# Autodesk Inventor assembly: LEG_MIR_MIR1
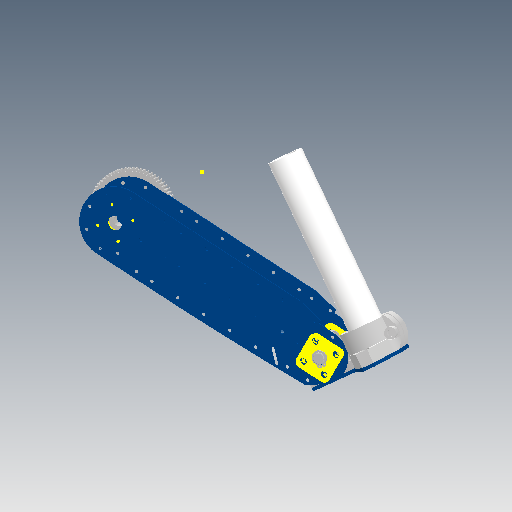
[picture p0: Inventor's stored thumbnail of the model, 512x512]
Saved by Autodesk Inventor 2020.5 (Build 245400000, 400)
## iProperties
Created: 2022-10-31
Part Number: LEG_MIR_MIR1
Document SubType Name: Assembly
Designer: kanazawakotaro
Author: Administrator
## Documents named in this file (12)
- C:\Users\Administrator\Documents\kamuy2\kamuy2\LEG_MIR_MIR1.iam
- C:\Users\Administrator\Documents\kamuy2\kamuy2\Parts\Part2_MIR_MIR_MIR1.ipt
- C:\Users\Administrator\Documents\kamuy2\kamuy2\Parts\GEABP1.0-70-10-A-19-KFC30-K3_Autodesk_Inventor_2020_20221114\AIS2020\GEABP1_0-70-10-A-19-KFC30-K3_MIR_MIR_MIR1.iam
- C:\Users\Administrator\Documents\kamuy2\kamuy2\Parts\PIJX30-20-150_Autodesk_Inventor_2020_20221115\PIJX30-20-150_MIR_MIR_MIR1.ipt
- C:\Users\Administrator\Documents\kamuy2\kamuy2\Parts\C-SHA10_Autodesk_Inventor_2020_20221104\AIS2020\C-SHA10_MIR_MIR_MIR1.iam
- C:\Users\Administrator\Documents\kamuy2\kamuy2\Part16_MIR_MIR_MIR1.ipt
- C:\Users\Administrator\Documents\kamuy2\kamuy2\Parts\HTPA30S3M060-A-N10_Autodesk_Inventor_2020_20221115\AIS2020\HTPA30S3M060-A-N10_MIR_MIR_MIR1.iam
- C:\Users\Administrator\Documents\kamuy2\kamuy2\Part20_MIR_MIR_MIR1.ipt
- C:\Users\Administrator\Documents\kamuy2\kamuy2\Parts\SMYHF30_STEP_AP203AP214\SMYHF30_203_MIR_MIR_MIR1.ipt
- C:\Users\Administrator\Documents\kamuy2\kamuy2\Part22_MIR_MIR_MIR1.ipt
- C:\Users\Administrator\Documents\kamuy2\kamuy2\Parts\RORPOS20-L30_Autodesk_Inventor_2020_20221117\AIS2020\RORPOS20-L30_MIR_MIR_MIR1.iam
- C:\Users\Administrator\Documents\kamuy2\kamuy2\Parts\NSFMRRA10-74-B3-S3-KC31.5-A11_Autodesk_Inventor_2020_20221116\AIS2020\NSFMRRA10-74-B3-S3-KC31_5-A11(000_000)_MIR_MIR_MIR1.iam
## Components (16 placed, 11 different names)
1. Part2_MIR_MIR_MIR1:1
2. GEABP1_0-70-10-A-19-KFC30-K3_MIR_MIR_MIR1:1 [sub-assembly] — フラッシュ:123
3. PIJX30-20-150_MIR_MIR_MIR1:1 — メイト:244, メイト:245
4. C-SHA10_MIR_MIR_MIR1:1 [sub-assembly] — フラッシュ:131, フラッシュ:89, メイト:235, メイト:249, フラッシュ:133, メイト:264
5. C-SHA10_MIR_MIR_MIR1:2 [sub-assembly] — フラッシュ:131, フラッシュ:89, メイト:237, メイト:250
6. Part16_MIR_MIR_MIR1:1 — フラッシュ:96, フラッシュ:122, メイト:236
7. Part16_MIR_MIR_MIR1:2 — フラッシュ:96, メイト:219, メイト:164, メイト:230
8. Part16_MIR_MIR_MIR1:3 — フラッシュ:122, メイト:219, メイト:234, フラッシュ:139, メイト:252
9. HTPA30S3M060-A-N10_MIR_MIR_MIR1:1 [sub-assembly] — フラッシュ:138, メイト:263
10. HTPA30S3M060-A-N10_MIR_MIR_MIR1:2 [sub-assembly] — フラッシュ:138, メイト:164
11. Part20_MIR_MIR_MIR1:1 — メイト:237, メイト:236, フラッシュ:123, メイト:265, メイト:66, メイト:68
12. Part20_MIR_MIR_MIR1:2 — メイト:265, メイト:235, メイト:234, メイト:230, メイト:251, メイト:247, メイト:253, メイト:69
13. SMYHF30_203_MIR_MIR_MIR1:1 — メイト:244, メイト:246, フラッシュ:135, メイト:242
14. Part22_MIR_MIR_MIR1:1 — メイト:250, メイト:249, メイト:246, フラッシュ:135, メイト:245, メイト:242, フラッシュ:133
15. RORPOS20-L30_MIR_MIR_MIR1:1 [sub-assembly] — メイト:251, メイト:247
16. NSFMRRA10-74-B3-S3-KC31_5-A11(000_000)_MIR_MIR_MIR1:1 [sub-assembly] — メイト:264, メイト:263, メイト:253, フラッシュ:139, メイト:252, メイト:66, メイト:68, メイト:69
## Relationships (32: Mate 25, Flush 7)
- フラッシュ:131 [Flush]: C-SHA10_MIR_MIR_MIR1:1 ↔ C-SHA10_MIR_MIR_MIR1:2
- フラッシュ:89 [Flush]: C-SHA10_MIR_MIR_MIR1:1 ↔ C-SHA10_MIR_MIR_MIR1:2
- フラッシュ:96 [Flush]: Part16_MIR_MIR_MIR1:1 ↔ Part16_MIR_MIR_MIR1:2
- フラッシュ:122 [Flush]: Part16_MIR_MIR_MIR1:1 ↔ Part16_MIR_MIR_MIR1:3
- メイト:219 [Mate] (168 mm): Part16_MIR_MIR_MIR1:2 ↔ Part16_MIR_MIR_MIR1:3
- フラッシュ:138 [Flush]: HTPA30S3M060-A-N10_MIR_MIR_MIR1:1 ↔ HTPA30S3M060-A-N10_MIR_MIR_MIR1:2
- メイト:164 [Mate] (7 mm): Part16_MIR_MIR_MIR1:2 ↔ HTPA30S3M060-A-N10_MIR_MIR_MIR1:2
- メイト:237 [Mate] (6 mm): C-SHA10_MIR_MIR_MIR1:2 ↔ Part20_MIR_MIR_MIR1:1
- メイト:236 [Mate]: Part16_MIR_MIR_MIR1:1 ↔ Part20_MIR_MIR_MIR1:1
- フラッシュ:123 [Mate]: GEABP1_0-70-10-A-19-KFC30-K3_MIR_MIR_MIR1:1 ↔ Part20_MIR_MIR_MIR1:1
- メイト:265 [Mate]: Part20_MIR_MIR_MIR1:1 ↔ Part20_MIR_MIR_MIR1:2
- メイト:235 [Mate] (6 mm): C-SHA10_MIR_MIR_MIR1:1 ↔ Part20_MIR_MIR_MIR1:2
- メイト:234 [Mate]: Part16_MIR_MIR_MIR1:3 ↔ Part20_MIR_MIR_MIR1:2
- メイト:230 [Mate]: Part16_MIR_MIR_MIR1:2 ↔ Part20_MIR_MIR_MIR1:2
- メイト:244 [Mate]: PIJX30-20-150_MIR_MIR_MIR1:1 ↔ SMYHF30_203_MIR_MIR_MIR1:1
- メイト:250 [Mate]: C-SHA10_MIR_MIR_MIR1:2 ↔ Part22_MIR_MIR_MIR1:1
- メイト:249 [Mate]: C-SHA10_MIR_MIR_MIR1:1 ↔ Part22_MIR_MIR_MIR1:1
- メイト:246 [Mate]: SMYHF30_203_MIR_MIR_MIR1:1 ↔ Part22_MIR_MIR_MIR1:1
- フラッシュ:135 [Flush]: SMYHF30_203_MIR_MIR_MIR1:1 ↔ Part22_MIR_MIR_MIR1:1
- メイト:245 [Mate]: PIJX30-20-150_MIR_MIR_MIR1:1 ↔ Part22_MIR_MIR_MIR1:1
- メイト:242 [Mate]: SMYHF30_203_MIR_MIR_MIR1:1 ↔ Part22_MIR_MIR_MIR1:1
- フラッシュ:133 [Mate]: C-SHA10_MIR_MIR_MIR1:1 ↔ Part22_MIR_MIR_MIR1:1
- メイト:251 [Mate]: Part20_MIR_MIR_MIR1:2 ↔ RORPOS20-L30_MIR_MIR_MIR1:1
- メイト:247 [Mate] (2.5 mm): Part20_MIR_MIR_MIR1:2 ↔ RORPOS20-L30_MIR_MIR_MIR1:1
- メイト:264 [Mate]: C-SHA10_MIR_MIR_MIR1:1 ↔ NSFMRRA10-74-B3-S3-KC31_5-A11(000_000)_MIR_MIR_MIR1:1
- メイト:263 [Mate]: HTPA30S3M060-A-N10_MIR_MIR_MIR1:1 ↔ NSFMRRA10-74-B3-S3-KC31_5-A11(000_000)_MIR_MIR_MIR1:1
- メイト:253 [Mate]: Part20_MIR_MIR_MIR1:2 ↔ NSFMRRA10-74-B3-S3-KC31_5-A11(000_000)_MIR_MIR_MIR1:1
- フラッシュ:139 [Flush] (-3 mm): Part16_MIR_MIR_MIR1:3 ↔ NSFMRRA10-74-B3-S3-KC31_5-A11(000_000)_MIR_MIR_MIR1:1
- メイト:252 [Mate]: Part16_MIR_MIR_MIR1:3 ↔ NSFMRRA10-74-B3-S3-KC31_5-A11(000_000)_MIR_MIR_MIR1:1
- メイト:66 [Mate]: Part20_MIR_MIR_MIR1:1 ↔ NSFMRRA10-74-B3-S3-KC31_5-A11(000_000)_MIR_MIR_MIR1:1
- メイト:68 [Mate]: Part20_MIR_MIR_MIR1:1 ↔ NSFMRRA10-74-B3-S3-KC31_5-A11(000_000)_MIR_MIR_MIR1:1
- メイト:69 [Mate]: Part20_MIR_MIR_MIR1:2 ↔ NSFMRRA10-74-B3-S3-KC31_5-A11(000_000)_MIR_MIR_MIR1:1
